# Autodesk Inventor assembly: assembage générale
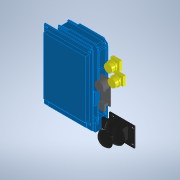
[picture p0: Inventor's stored thumbnail of the model, 180x180]
Saved by Autodesk Inventor 2020 (Build 240168000, 168)
## iProperties
Created: 2020-01-17
Part Number: assembage générale
Document SubType Name: Assembly
Designer: Manuel Enzo
Author: Manuel Enzo
## Documents named in this file (7)
- C:\Users\enzom\Desktop\Projet arduino\Modélisation\assembage générale.iam
- C:\Users\enzom\Desktop\Projet arduino\Modélisation\Couvercle supérieur.ipt
- C:\Users\enzom\Desktop\Projet arduino\Modélisation\Couvercle inférieur.ipt
- C:\Users\enzom\Desktop\Projet arduino\Modélisation\Assemblage carte_ecran.iam
- C:\Users\enzom\Desktop\Projet arduino\Modélisation\Joystick.ipt
- C:\Users\enzom\Desktop\Projet arduino\Modélisation\Bouton.ipt
- C:\Users\enzom\Desktop\Projet arduino\Modélisation\Buzzer.ipt
## Components (7 placed, 6 different names)
1. Couvercle supérieur:1 — Placage:1, Placage:2, Placage:3, Placage:4, Placage:5, Placage:6, Placage:7, Placage:8, Placage:9, Placage:10, Affleurement:1
2. Couvercle inférieur:1 — Placage:1, Placage:2, Placage:11, Placage:12, Placage:13
3. Assemblage carte_ecran:1 [sub-assembly] — Placage:3, Placage:4, Placage:5
4. Joystick:1 — Placage:10, Affleurement:1, Placage:11
5. Bouton:1 — Placage:6, Placage:7
6. Bouton:2 — Placage:8, Placage:9
7. Buzzer:1 — Placage:12, Placage:13
## Relationships (14: Mate 13, Flush 1)
- Placage:1 [Mate]: Couvercle supérieur:1 ↔ Couvercle inférieur:1
- Placage:2 [Mate]: Couvercle supérieur:1 ↔ Couvercle inférieur:1
- Placage:3 [Mate]: Couvercle supérieur:1 ↔ Assemblage carte_ecran:1
- Placage:4 [Mate]: Couvercle supérieur:1 ↔ Assemblage carte_ecran:1
- Placage:5 [Mate]: Couvercle supérieur:1 ↔ Assemblage carte_ecran:1
- Placage:6 [Mate]: Couvercle supérieur:1 ↔ Bouton:1
- Placage:7 [Mate]: Couvercle supérieur:1 ↔ Bouton:1
- Placage:8 [Mate]: Couvercle supérieur:1 ↔ Bouton:2
- Placage:9 [Mate]: Couvercle supérieur:1 ↔ Bouton:2
- Placage:10 [Mate]: Couvercle supérieur:1 ↔ Joystick:1
- Affleurement:1 [Flush]: Couvercle supérieur:1 ↔ Joystick:1
- Placage:11 [Mate]: Couvercle inférieur:1 ↔ Joystick:1
- Placage:12 [Mate]: Couvercle inférieur:1 ↔ Buzzer:1
- Placage:13 [Mate]: Couvercle inférieur:1 ↔ Buzzer:1
